# Autodesk Inventor assembly: assembily_v2
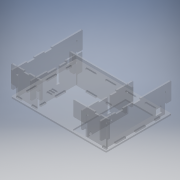
[picture p0: Inventor's stored thumbnail of the model, 180x180]
Saved by Autodesk Inventor 2017.2 (Build 212233000, 233)
## iProperties
Created: 2017-06-09
Part Number: assembily_v2
Document SubType Name: Assembly
Designer: SandeepSH
Author: SandeepSH
## Documents named in this file (8)
- C:\Users\SandeepSH\Dropbox\MSC\Project\inventor\lcv1\assembily_v2.iam
- C:\Users\SandeepSH\Dropbox\MSC\Project\inventor\lcv1\base_v2.ipt
- C:\Users\SandeepSH\Dropbox\MSC\Project\inventor\lcv1\cham_right_v2.ipt
- C:\Users\SandeepSH\Dropbox\MSC\Project\inventor\lcv1\cham_back_v2.ipt
- C:\Users\SandeepSH\Dropbox\MSC\Project\inventor\lcv1\front_right_v2.ipt
- C:\Users\SandeepSH\Dropbox\MSC\Project\inventor\lcv1\cham_left_v2.ipt
- C:\Users\SandeepSH\Dropbox\MSC\Project\inventor\lcv1\front_left_v2.ipt
- C:\Users\SandeepSH\Dropbox\MSC\Project\inventor\lcv1\side_v2.ipt
## Components (8 placed, 7 different names)
1. base_v2:1 — Mate:1, Mate:2, Mate:3, Mate:6, Mate:7, Mate:8, Mate:9, Mate:10, Mate:11, Mate:12, Mate:13, Mate:14, Mate:15
2. front_right_v2:1 — Mate:1, Mate:6
3. cham_back_v2:1 — Mate:2, Mate:3, Mate:4, Mate:5, Mate:7
4. cham_right_v2:1 — Mate:4, Mate:5
5. cham_left_v2:1 — Mate:8, Mate:9
6. front_left_v2:1 — Mate:10, Mate:11
7. side_v2:1 — Mate:12, Mate:13
8. side_v2:2 — Mate:14, Mate:15
## Relationships (15: Mate 15)
- Mate:1: base_v2:1 ↔ front_right_v2:1
- Mate:2: base_v2:1 ↔ cham_back_v2:1
- Mate:3: base_v2:1 ↔ cham_back_v2:1
- Mate:4: cham_back_v2:1 ↔ cham_right_v2:1
- Mate:5: cham_back_v2:1 ↔ cham_right_v2:1
- Mate:6: base_v2:1 ↔ front_right_v2:1
- Mate:7: base_v2:1 ↔ cham_back_v2:1
- Mate:8: base_v2:1 ↔ cham_left_v2:1
- Mate:9: base_v2:1 ↔ cham_left_v2:1
- Mate:10: base_v2:1 ↔ front_left_v2:1
- Mate:11: base_v2:1 ↔ front_left_v2:1
- Mate:12: base_v2:1 ↔ side_v2:1
- Mate:13: base_v2:1 ↔ side_v2:1
- Mate:14: base_v2:1 ↔ side_v2:2
- Mate:15: base_v2:1 ↔ side_v2:2
